# Autodesk Inventor assembly: FingerBase_Assembly
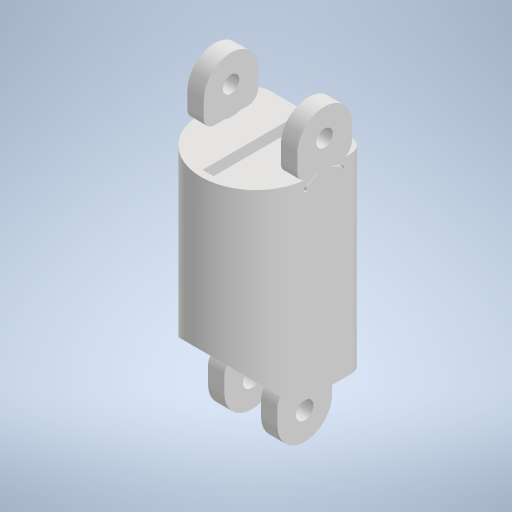
[picture p0: Inventor's stored thumbnail of the model, 512x512]
Saved by Autodesk Inventor 2023 (Build 270158000, 158)
## iProperties
Created: 2023-04-11
Part Number: FingerBase_Assembly
Document SubType Name: Assembly
Designer: 1SENADI
Author: 1SENADI
## Documents named in this file (4)
- C:\Users\1SENADI\Desktop\FingerBase_Assembly.iam
- C:\Users\1SENADI\Downloads\BaseKnuckle.ipt
- C:\Users\1SENADI\Downloads\Knuckle Attachment DirectInsert.ipt
- C:\Users\1SENADI\Downloads\Knuckle Attachment SMALL HOLE.ipt
## Components (5 placed, 3 different names)
1. BaseKnuckle:1 — Mate:1, Mate:2, Mate:3, Mate:4, Mate:5, Mate:6, Mate:7, Mate:8, Mate:9
2. Knuckle Attachment SMALL HOLE:1 — Mate:1, Mate:2, Mate:3
3. Knuckle Attachment SMALL HOLE:2 — Mate:4
4. Knuckle Attachment DirectInsert:3 — Mate:8, Mate:9
5. Knuckle Attachment DirectInsert:4 — Mate:5, Mate:6, Mate:7
## Relationships (9: Mate 9)
- Mate:1: BaseKnuckle:1 ↔ Knuckle Attachment SMALL HOLE:1
- Mate:2: BaseKnuckle:1 ↔ Knuckle Attachment SMALL HOLE:1
- Mate:3: BaseKnuckle:1 ↔ Knuckle Attachment SMALL HOLE:1
- Mate:4: BaseKnuckle:1 ↔ Knuckle Attachment SMALL HOLE:2
- Mate:5: BaseKnuckle:1 ↔ Knuckle Attachment DirectInsert:4
- Mate:6: BaseKnuckle:1 ↔ Knuckle Attachment DirectInsert:4
- Mate:7: BaseKnuckle:1 ↔ Knuckle Attachment DirectInsert:4
- Mate:8: BaseKnuckle:1 ↔ Knuckle Attachment DirectInsert:3
- Mate:9: BaseKnuckle:1 ↔ Knuckle Attachment DirectInsert:3
